# Autodesk Inventor assembly: 조립품1
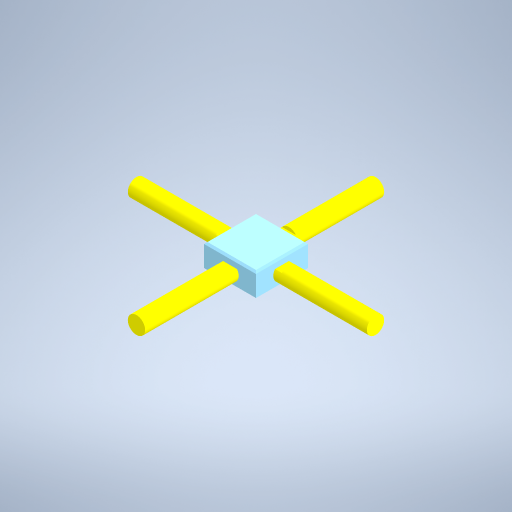
[picture p0: Inventor's stored thumbnail of the model, 512x512]
Saved by Autodesk Inventor 2023 (Build 270158000, 158)
## iProperties
Created: 2022-10-29
Part Number: 조립품1
Document SubType Name: Assembly
Designer: 전상현
Author: 전상현
## Documents named in this file (3)
- C:\Users\전상현\Documents\Inventor\lecture\moodlight\출력\조립품1.iam
- C:\Users\전상현\Documents\Inventor\lecture\moodlight\교육용\몸통.ipt
- C:\Users\전상현\Documents\Inventor\lecture\moodlight\교육용\팔.ipt
## Components (5 placed, 2 different names)
1. 몸통:1 — 메이트:1, 메이트:2, 플러쉬:1, 메이트:3, 메이트:4, 메이트:5
2. 팔:1 — 메이트:3, 메이트:4, 메이트:5
3. 팔:2
4. 팔:3
5. 팔:4
## Component patterns: (4 elements, first: 팔:1)
## Relationships (6: Mate 5, Flush 1)
- 메이트:1 [Mate]: 몸통:1
- 메이트:2 [Mate]: 몸통:1
- 플러쉬:1 [Flush]: 몸통:1
- 메이트:3 [Mate]: 몸통:1 ↔ 팔:1
- 메이트:4 [Mate]: 몸통:1 ↔ 팔:1
- 메이트:5 [Mate]: 몸통:1 ↔ 팔:1
